# Autodesk Inventor assembly: NCME075-0400.step
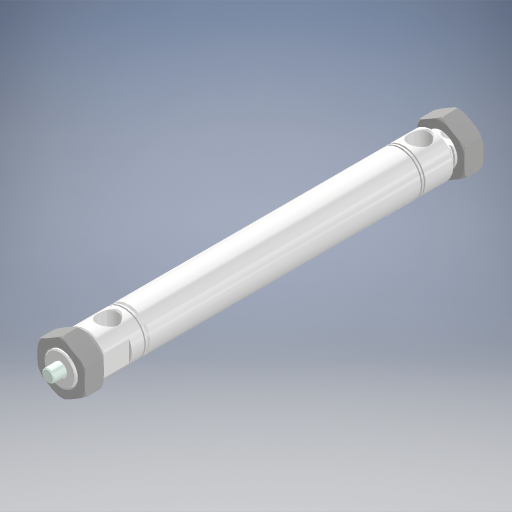
[picture p0: Inventor's stored thumbnail of the model, 512x512]
Saved by Autodesk Inventor 2024.2 (Build 282272000, 272)
## iProperties
Created: 2016-06-17
Part Number: NCME075-0400.step
Description: STEP AP214
Document SubType Name: Assembly
Designer: rohan
Sending System: SolidWorks 2016
Preprocessor: SwSTEP 2.0
Title: NCME075-0400.step.step
Author: Windows User
Revision Number: ANY
## Documents named in this file (4)
- C:\Users\rohan\OneDrive - Hillsborough County Public Schools\Robotics\FIRST-Robotics-Competition\Crescendo\Minotaur-Crescendo-Robot\Motion\Cylinders\ANDYMARK-4in-Cylinder.iam
- C:\Users\rohan\OneDrive - Hillsborough County Public Schools\Robotics\FIRST-Robotics-Competition\Crescendo\Minotaur-Crescendo-Robot\Motion\Cylinders\am-2034_4\NCME075-0400.step_NCM-Body_075E.ipt
- C:\Users\rohan\OneDrive - Hillsborough County Public Schools\Robotics\FIRST-Robotics-Competition\Crescendo\Minotaur-Crescendo-Robot\Motion\Cylinders\am-2034_4\NCME075-0400.step_NCM-Rod_075.ipt
- C:\Users\rohan\OneDrive - Hillsborough County Public Schools\Robotics\FIRST-Robotics-Competition\Crescendo\Minotaur-Crescendo-Robot\Motion\Cylinders\am-2034_4\NCME075-0400.step_NCM-Nut_075.ipt
## Components (4 placed, 4 different names)
1. NCME075-0400.step_NCM-Body_075E_1 — Mate:1, Flush:1, Mate:2, Flush:2, Cylindrical:1
2. NCME075-0400.step_NCM-Rod_075_2 — Cylindrical:1
3. NCME075-0400.step_NCM-Nut_075_3 — Mate:1, Flush:1
4. NCME075-0400.step_NCM-Nut_075_4 — Mate:2, Flush:2
## Relationships (5: Mate 2, Flush 2, CylindricalJoint 1)
- Mate:1: NCME075-0400.step_NCM-Body_075E_1 ↔ NCME075-0400.step_NCM-Nut_075_3
- Flush:1 (0.666 mm): NCME075-0400.step_NCM-Body_075E_1 ↔ NCME075-0400.step_NCM-Nut_075_3
- Mate:2: NCME075-0400.step_NCM-Body_075E_1 ↔ NCME075-0400.step_NCM-Nut_075_4
- Flush:2 (2.286 mm): NCME075-0400.step_NCM-Body_075E_1 ↔ NCME075-0400.step_NCM-Nut_075_4
- Cylindrical:1: NCME075-0400.step_NCM-Body_075E_1 ↔ NCME075-0400.step_NCM-Rod_075_2
